# Autodesk Inventor assembly: krzyzyk
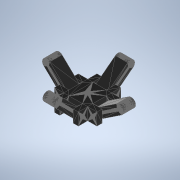
[picture p0: Inventor's stored thumbnail of the model, 180x180]
Saved by Autodesk Inventor 2022.3 (Build 263350000, 350)
## iProperties
Created: 2023-06-03
Part Number: krzyzyk
Document SubType Name: Assembly
Designer: komputer
Author: komputer
## Documents named in this file (3)
- C:\Users\komputer\Documents\Inventor\chwytak\krzyzyk.iam
- C:\Users\komputer\Documents\Inventor\chwytak\ArmMuscle.ipt
- C:\Users\komputer\Documents\Inventor\chwytak\GripperMotorHinges.ipt
## Components (5 placed, 2 different names)
1. ArmMuscle:1 — Mate:3, Mate:4
2. ArmMuscle:2 — Mate:1, Mate:2
3. ArmMuscle:3 — Mate:7, Mate:8
4. ArmMuscle:4 — Mate:5, Mate:6
5. GripperMotorHinges:1 — Mate:1, Mate:2, Mate:3, Mate:4, Mate:5, Mate:6, Mate:7, Mate:8
## Relationships (8: Mate 8)
- Mate:1 (0.5 mm): ArmMuscle:2 ↔ GripperMotorHinges:1
- Mate:2: ArmMuscle:2 ↔ GripperMotorHinges:1
- Mate:3: ArmMuscle:1 ↔ GripperMotorHinges:1
- Mate:4 (0.5 mm): ArmMuscle:1 ↔ GripperMotorHinges:1
- Mate:5 (0.5 mm): ArmMuscle:4 ↔ GripperMotorHinges:1
- Mate:6: ArmMuscle:4 ↔ GripperMotorHinges:1
- Mate:7: ArmMuscle:3 ↔ GripperMotorHinges:1
- Mate:8 (0.5 mm): ArmMuscle:3 ↔ GripperMotorHinges:1
